# Autodesk Inventor assembly: Rückplatte mit LED
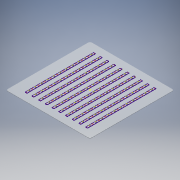
[picture p0: Inventor's stored thumbnail of the model, 180x180]
Saved by Autodesk Inventor 2019 (Build 230136000, 136)
## iProperties
Created: 2018-10-19
Part Number: Rückplatte mit LED
Material: Generisch
Document SubType Name: Assembly
Designer: Roger
Author: Roger
## Documents named in this file (3)
- C:\Users\Roger\Dropbox\Uhr\Rückplatte mit LED.iam
- C:\Users\Roger\Dropbox\Uhr\Rückplatte.ipt
- C:\Users\Roger\Dropbox\Uhr\LED_Strip.iam
## Components (11 placed, 2 different names)
1. Rückplatte:1 — Passend:1, Fluchtend:1, Fluchtend:2
2. LED_Strip:1 [sub-assembly] — Passend:1, Fluchtend:1, Fluchtend:2
3. LED_Strip:2 [sub-assembly]
4. LED_Strip:3 [sub-assembly]
5. LED_Strip:4 [sub-assembly]
6. LED_Strip:5 [sub-assembly]
7. LED_Strip:6 [sub-assembly]
8. LED_Strip:7 [sub-assembly]
9. LED_Strip:8 [sub-assembly]
10. LED_Strip:9 [sub-assembly]
11. LED_Strip:10 [sub-assembly]
## Component patterns: (10 elements, first: LED_Strip:1)
## Relationships (3: Flush 2, Mate 1)
- Passend:1 [Mate]: Rückplatte:1 ↔ LED_Strip:1
- Fluchtend:1 [Flush] (-60 mm): Rückplatte:1 ↔ LED_Strip:1
- Fluchtend:2 [Flush] (41.685 mm): Rückplatte:1 ↔ LED_Strip:1
